# Autodesk Inventor assembly: Differential Swerve Drive V3
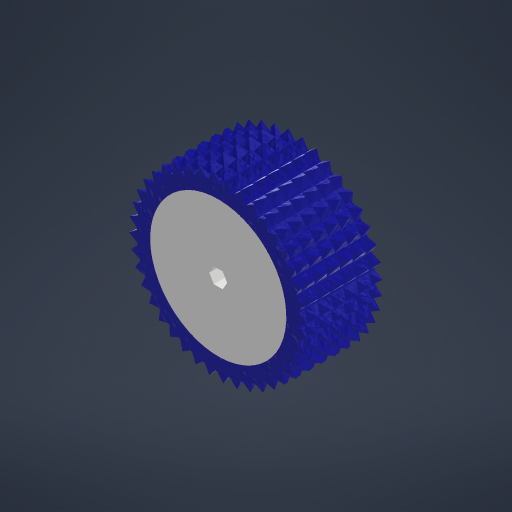
[picture p0: Inventor's stored thumbnail of the model, 512x512]
Saved by Autodesk Inventor 2024 (Build 280153000, 153)
## iProperties
Created: 2023-09-09
Part Number: Differential Swerve Drive V3
Document SubType Name: Assembly
Designer: izack
Author: izack
## Documents named in this file (3)
- C:\Users\izack\Robotics\CAD\Custom-Modules-CAD\Differential Swerve Drive V3.iam
- C:\Users\izack\Robotics\CAD\Custom-Modules-CAD\60mm Wheel Rim.ipt
- C:\Users\izack\Robotics\CAD\Custom-Modules-CAD\60mm Wheel Tire Tread.ipt
## Components (2 placed, 2 different names)
1. 60mm Wheel Rim:1 — Flush:1
2. 60mm Wheel Tire Tread:1 — Flush:1
## Relationships (1: Flush 1)
- Flush:1: 60mm Wheel Rim:1 ↔ 60mm Wheel Tire Tread:1
